# Autodesk Inventor assembly: LegLowerBackLinkUnit
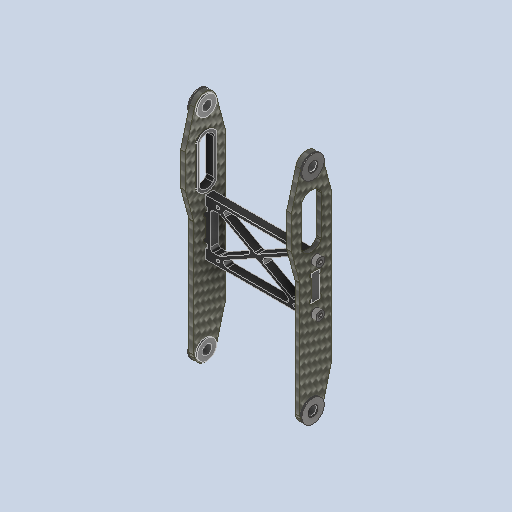
[picture p0: Inventor's stored thumbnail of the model, 512x512]
Saved by Autodesk Inventor 2024.2 (Build 282272000, 272)
## iProperties
Created: 2024-01-06
Part Number: LegLowerBackLinkUnit
Document SubType Name: Assembly
Designer: Masato Kubotera
Mass: 40.5776 g
Surface Area: 239.681 cm^2
Volume: 21.0227 cm^3
Density: 1.93018 g/cm^3
Author: Masato Kubotera
## Documents named in this file (3)
- C:\Users\masato\OneDrive - Chiba Institute of Technology\CIT Brains\RoboCup2024\Mechanic\SUSTAINA-OP2-DEV\NativeFiles\Boby\LowerLimb\Legs\Links\LegLowerBackLinkUnit.iam
- C:\Users\masato\OneDrive - Chiba Institute of Technology\CIT Brains\RoboCup2024\Mechanic\SUSTAINA-OP2-DEV\NativeFiles\Boby\CommonDesignedComponents\SliderProtectionFrame.ipt
- C:\Users\masato\OneDrive - Chiba Institute of Technology\CIT Brains\RoboCup2024\Mechanic\SUSTAINA-OP2-DEV\NativeFiles\Boby\LowerLimb\Legs\Links\LegBackLinkUnitBase.iam
## Components (2 placed, 2 different names)
1. LegBackLinkUnitBase:1 [sub-assembly] — Flush:1, Mate:3, Mate:4, Insert:1, Insert:2
2. SliderProtectionFrame:2 — Insert:1, Insert:2
## Relationships (5: Mate 2, Insert 2, Flush 1)
- Flush:1: LegBackLinkUnitBase:1
- Mate:3: LegBackLinkUnitBase:1
- Mate:4: LegBackLinkUnitBase:1
- Insert:1: LegBackLinkUnitBase:1 ↔ SliderProtectionFrame:2
- Insert:2: LegBackLinkUnitBase:1 ↔ SliderProtectionFrame:2
